# Autodesk Inventor assembly: Cartesian2_YAssembly
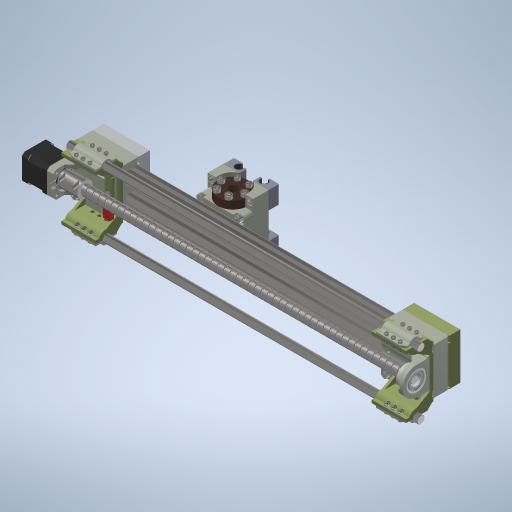
[picture p0: Inventor's stored thumbnail of the model, 512x512]
Saved by Autodesk Inventor 2024 (Build 280153000, 153)
## iProperties
Created: 2020-08-17
Part Number: Cartesian2_YAssembly
Material: Ogólny
Document SubType Name: Assembly
Designer: invin
Mass: 4227.11 g
Surface Area: 5602.37 cm^2
Volume: 1262.4 cm^3
Density: 3.34848 g/cm^3
Author: invin
## Documents named in this file (27)
- D:\@home\mikoma\Dokumenty\DR\CartesianRobotsDigitalTwin\model\Workspaces\Obszar roboczy\assembly_v3\Y\Y.iam
- D:\@home\mikoma\Dokumenty\DR\CartesianRobotsDigitalTwin\model\Workspaces\Obszar roboczy\content\item\item_0037003_Profile_5_20x20_L=564_1.ipt
- D:\@home\mikoma\Dokumenty\DR\CartesianRobotsDigitalTwin\model\Workspaces\Obszar roboczy\content\manipulatorSharedParts\Cartesian1_12mm_Rod.ipt
- D:\@home\mikoma\Dokumenty\DR\CartesianRobotsDigitalTwin\model\Workspaces\Obszar roboczy\content\manipulatorSharedParts\Cartesian2_BallBearing_25x37x7.ipt
- D:\@home\mikoma\Dokumenty\DR\CartesianRobotsDigitalTwin\model\Workspaces\Obszar roboczy\assembly_v3\Y\Cartesian1_X_RodCover.ipt
- D:\@home\mikoma\Dokumenty\DR\CartesianRobotsDigitalTwin\model\Workspaces\Obszar roboczy\content\nema17\Nema17 Stepper Motor.ipt
- D:\@home\mikoma\Dokumenty\DR\CartesianRobotsDigitalTwin\model\Workspaces\Obszar roboczy\content\manipulatorSharedParts\Cartesian1_12_12_Clutch.ipt
- D:\@home\mikoma\Dokumenty\DR\CartesianRobotsDigitalTwin\model\Workspaces\Obszar roboczy\content\manipulatorSharedParts\Cartesian1_BallScrew.ipt
- D:\@home\mikoma\Dokumenty\DR\CartesianRobotsDigitalTwin\model\Workspaces\Obszar roboczy\content\igus\WJ200UM_01_10_1.ipt
- D:\@home\mikoma\Dokumenty\DR\CartesianRobotsDigitalTwin\model\Workspaces\Obszar roboczy\assembly_v3\Y\YSub1.iam
- D:\@home\mikoma\Dokumenty\DR\CartesianRobotsDigitalTwin\model\Workspaces\Obszar roboczy\assembly_v3\Y\YSub2.iam
- D:\@home\mikoma\Dokumenty\DR\CartesianRobotsDigitalTwin\model\Workspaces\Obszar roboczy\assembly_v3\Y\YItemEndCover.ipt
- D:\@home\mikoma\Dokumenty\DR\CartesianRobotsDigitalTwin\model\Workspaces\Obszar roboczy\assembly_v3\Y\YCarriage.ipt
- D:\@home\mikoma\Dokumenty\DR\CartesianRobotsDigitalTwin\model\Workspaces\Obszar roboczy\assembly_v3\Y\YCarriageNut.ipt
- D:\@home\mikoma\Dokumenty\DR\CartesianRobotsDigitalTwin\model\Workspaces\Obszar roboczy\assembly_v3\Y\YItemEnd.ipt
- D:\@home\mikoma\Dokumenty\DR\CartesianRobotsDigitalTwin\model\Workspaces\Obszar roboczy\assembly_v3\Y\YItemEndCoverConnector.ipt
- D:\@home\mikoma\Dokumenty\DR\CartesianRobotsDigitalTwin\model\Workspaces\Obszar roboczy\content\manipulatorSharedParts\endCup.ipt
- D:\@home\mikoma\Dokumenty\DR\CartesianRobotsDigitalTwin\model\Workspaces\Obszar roboczy\CC\pl-PL\ISO 4762(1)\DIN EN ISO 4762 - M5 x 50.ipt
- D:\@home\mikoma\Dokumenty\DR\CartesianRobotsDigitalTwin\model\Workspaces\Obszar roboczy\CC\pl-PL\ISO 4762(1)\DIN EN ISO 4762 - M6 x 55.ipt
- D:\@home\mikoma\Dokumenty\DR\CartesianRobotsDigitalTwin\model\Workspaces\Obszar roboczy\CC\pl-PL\ISO 4032(2)\ISO 4032 - M6 - ISO.ipt
- D:\@home\mikoma\Dokumenty\DR\CartesianRobotsDigitalTwin\model\Workspaces\Obszar roboczy\CC\pl-PL\ISO 4762(1)\DIN EN ISO 4762 - M6 x 30.ipt
- D:\@home\mikoma\Dokumenty\DR\CartesianRobotsDigitalTwin\model\Workspaces\Obszar roboczy\content\item\item_0037006_Wpust_przesuwny_5_St_M4_1.ipt
- D:\@home\mikoma\Dokumenty\DR\CartesianRobotsDigitalTwin\model\Workspaces\Obszar roboczy\CC\pl-PL\DIN 7984\DIN 7984 - M4 x 14.ipt
- D:\@home\mikoma\Dokumenty\DR\CartesianRobotsDigitalTwin\model\Workspaces\Obszar roboczy\CC\pl-PL\ISO 4032(2)\ISO 4032 - M5 - ISO.ipt
- D:\@home\mikoma\Dokumenty\DR\CartesianRobotsDigitalTwin\model\Workspaces\Obszar roboczy\content\manipulatorSharedParts\Connector_female.ipt
- D:\@home\mikoma\Dokumenty\DR\CartesianRobotsDigitalTwin\model\Workspaces\Obszar roboczy\CC\pl-PL\ISO 4032(2)\ISO 4032 - M3 - ISO.ipt
- D:\@home\mikoma\Dokumenty\DR\CartesianRobotsDigitalTwin\model\Workspaces\Obszar roboczy\CC\pl-PL\ISO 4762(1)\DIN EN ISO 4762 - M3 x 12.ipt
## Components (115 placed, 26 different names)
1. YSub1:1 [sub-assembly] — Zestawiający:1, Kąt:1, Zestawiający:6, Zestawiający:7, Zestawiający:9, Zestawiający:10, Zestawiający:13, Zestawiający:32, Zestawiający:33, Zestawiający:34, Zestawiający:35, Zestawiający:36, Zestawiający:37, Zestawiający:44, Kąt:3, Zestawiający:45, Zestawiające:57, Zestawiające:75, Równoległe:14, Równoległe:15, Zestawiające:82, Zestawiające:83, Zestawiające:84, Zestawiające:85, Zestawiające:86, Zestawiające:87, Zestawiające:88, Zestawiające:89, Zestawiające:90, Równoległe:20, Równoległe:21, Zestawiające:174, Zestawiające:179, Kątowe:21, Kątowe:24
2. YSub2:1 [sub-assembly] — Zestawiający:1, Kąt:1, Zestawiający:12, Zestawiający:24, Zestawiający:25, Zestawiający:26, Zestawiający:27, Zestawiający:28, Zestawiający:29, Zestawiający:30, Zestawiający:31, Zestawiające:50, Równoległe:3, Zestawiające:91, Zestawiające:92, Zestawiające:93, Zestawiające:94, Zestawiające:95, Zestawiające:96, Zestawiające:97, Zestawiające:98, Zestawiające:184, Kątowe:22, Zestawiające:188, Kątowe:23
3. YItemEnd:1 — Zestawiające:50, Zestawiające:52, Równoległe:3, Zestawiające:53, Równoległe:4, Równoległe:5, Zestawiające:55, Zestawiające:56
4. item_0037003_Profile_5_20x20_L=564_1:1 — Zestawiający:9, Zestawiający:10, Zestawiające:56, Kątowe:10, Zestawiające:145, Kątowe:11, Zestawiające:149
5. item_0037003_Profile_5_20x20_L=564_1:2 — Zestawiający:6, Zestawiający:7, Zestawiające:52, Zestawiające:55, Zestawiające:57, Zestawiające:58, Zestawiające:138, Kątowe:8, Kątowe:9, Zestawiające:141
6. Cartesian1_12mm_Rod:1 — Zestawiający:13, Równoległe:21
7. Cartesian1_12mm_Rod:2 — Zestawiający:12, Równoległe:20
8. Cartesian2_BallBearing_25x37x7:1 — Zestawiający:24, Zestawiający:25, Zestawiające:78, Zestawiające:80, Zestawiające:81
9. Cartesian1_X_RodCover:1 — Zestawiający:26, Zestawiający:27, Zestawiający:28, Zestawiające:181, Zestawiające:182
10. Cartesian1_X_RodCover:2 — Zestawiający:29, Zestawiający:30, Zestawiający:31, Zestawiające:186, Zestawiające:187
11. Cartesian1_X_RodCover:3 — Zestawiający:32, Zestawiający:33, Zestawiający:34
12. Cartesian1_X_RodCover:4 — Zestawiający:35, Zestawiający:36, Zestawiający:37, Zestawiające:176, Zestawiające:177
13. Nema17 Stepper Motor:2 — Zestawiający:44, Kąt:3, Zestawiający:45, Zestawiający:46, Zestawiający:47
14. Cartesian1_12_12_Clutch:1 — Zestawiający:46, Zestawiający:47, Zestawiający:48, Zestawiający:49
15. Cartesian1_BallScrew:1 — Zestawiający:48, Zestawiający:49
16. YItemEndCover:1 — Zestawiające:53, Równoległe:4, Równoległe:5, Kątowe:12, Zestawiające:153, Kątowe:13, Zestawiające:155, Kątowe:14, Zestawiające:157, Kątowe:15, Zestawiające:159
17. YCarriage:1 — Zestawiające:58, Zestawiające:59, Zestawiające:61, Zestawiające:62, Zestawiające:63, Zestawiające:64, Zestawiające:65, Zestawiające:66, Zestawiające:67, Zestawiające:68, Zestawiające:69, Zestawiające:70, Zestawiające:71, Zestawiające:72, Zestawiające:73, Równoległe:13, Zestawiające:99, Zestawiające:111, Zestawiające:112, Zestawiające:113, Zestawiające:114, Zestawiające:115, Zestawiające:116, Zestawiające:117, Zestawiające:118, Zestawiające:119, Zestawiające:120, Zestawiające:121, Zestawiające:122, Zestawiające:123, Kątowe:4, Zestawiające:125, Zestawiające:127, Kątowe:5, Kątowe:6, Zestawiające:128, Kątowe:7, Zestawiające:130, Zestawiające:132, Zestawiające:133, Zestawiające:134, Zestawiające:135, Zestawiające:136, Zestawiające:137, Zestawiające:139, Zestawiające:140, Zestawiające:142, Zestawiające:143, Zestawiające:144, Zestawiające:146, Zestawiające:147, Zestawiające:148, Zestawiające:150, Zestawiające:151
18. YCarriageNut:1 — Zestawiające:59, Zestawiające:61, Zestawiające:82, Zestawiające:100, Zestawiające:101, Zestawiające:102, Zestawiające:103, Zestawiające:104, Zestawiające:105, Zestawiające:106, Zestawiające:107, Zestawiające:108, Zestawiające:109, Zestawiające:110
19. WJ200UM_01_10_1:1 — Zestawiające:62, Zestawiające:63, Zestawiające:64
20. WJ200UM_01_10_1:2 — Zestawiające:65, Zestawiające:66, Zestawiające:67
21. WJ200UM_01_10_1:3 — Zestawiające:68, Zestawiające:69, Zestawiające:70
22. WJ200UM_01_10_1:4 — Zestawiające:71, Zestawiające:72, Zestawiające:73
23. YItemEndCoverConnector:1 — Zestawiające:75, Równoległe:14, Równoległe:15, Zestawiające:79, Kątowe:16, Zestawiające:161, Kątowe:17, Zestawiające:163, Kątowe:18, Zestawiające:165, Kątowe:19, Zestawiające:167, Zestawiające:168, Zestawiające:169, Zestawiające:170
24. endCup:1 — Zestawiające:80, Zestawiające:81
25. DIN EN ISO 4762 M5 x 50:1 — Zestawiające:83, Zestawiające:84, Zestawiające:160
26. DIN EN ISO 4762 M5 x 50:2 — Zestawiające:85, Zestawiające:86, Zestawiające:166
27. DIN EN ISO 4762 M5 x 50:3 — Zestawiające:87, Zestawiające:88, Zestawiające:162
28. DIN EN ISO 4762 M5 x 50:4 — Zestawiające:89, Zestawiające:90, Zestawiające:164
29. DIN EN ISO 4762 M5 x 50:5 — Zestawiające:91, Zestawiające:95, Zestawiające:152
30. DIN EN ISO 4762 M5 x 50:6 — Zestawiające:92, Zestawiające:98, Zestawiające:158
31. DIN EN ISO 4762 M5 x 50:7 — Zestawiające:93, Zestawiające:96, Zestawiające:154
32. DIN EN ISO 4762 M5 x 50:8 — Zestawiające:94, Zestawiające:97, Zestawiające:156
33. DIN EN ISO 4762 M5 x 50:9 — Zestawiające:99, Zestawiające:100
34. DIN EN ISO 4762 M5 x 50:10 — Zestawiające:101, Zestawiające:102
35. DIN EN ISO 4762 M6 x 55:1 — Zestawiające:103, Zestawiające:107, Zestawiające:131
36. DIN EN ISO 4762 M6 x 55:2 — Zestawiające:111, Zestawiające:112
37. DIN EN ISO 4762 M6 x 55:3 — Zestawiające:104, Zestawiające:108, Zestawiające:129
38. DIN EN ISO 4762 M6 x 55:4 — Zestawiające:105, Zestawiające:110, Zestawiające:124
39. DIN EN ISO 4762 M6 x 55:5 — Zestawiające:106, Zestawiające:109, Zestawiające:123, Zestawiające:126
40. DIN EN ISO 4762 M6 x 55:6 — Zestawiające:113, Zestawiające:114
41. DIN EN ISO 4762 M6 x 55:7 — Zestawiające:115, Zestawiające:116
42. DIN EN ISO 4762 M6 x 55:8 — Zestawiające:117, Zestawiające:118
43. DIN EN ISO 4762 M6 x 55:9 — Zestawiające:119, Zestawiające:120
44. DIN EN ISO 4762 M6 x 55:10 — Zestawiające:121, Zestawiające:122
45. ISO 4032 M6:1 — Zestawiające:124, Kątowe:4, Zestawiające:125
46. ISO 4032 M6:2 — Zestawiające:126, Zestawiające:127, Kątowe:5
47. ISO 4032 M6:3 — Kątowe:6, Zestawiające:128, Zestawiające:129
48. ISO 4032 M6:4 — Kątowe:7, Zestawiające:130, Zestawiające:131
49. DIN EN ISO 4762 M6 x 30:1 — Zestawiające:132, Zestawiające:133
50. DIN EN ISO 4762 M6 x 30:2 — Zestawiające:134, Zestawiające:135
51. item_0037006_Wpust_przesuwny_5_St_M4_1:1 — Zestawiające:137, Zestawiające:138, Kątowe:8
52. DIN 7984 M4 x 14:1 — Zestawiające:136, Zestawiające:139
53. DIN 7984 M4 x 14:2 — Zestawiające:142, Zestawiające:143
54. item_0037006_Wpust_przesuwny_5_St_M4_1:2 — Zestawiające:140, Kątowe:9, Zestawiające:141
55. item_0037006_Wpust_przesuwny_5_St_M4_1:3 — Zestawiające:144, Kątowe:10, Zestawiające:145
56. DIN 7984 M4 x 14:3 — Zestawiające:146, Zestawiające:147
57. item_0037006_Wpust_przesuwny_5_St_M4_1:4 — Zestawiające:148, Kątowe:11, Zestawiające:149
58. DIN 7984 M4 x 14:4 — Zestawiające:150, Zestawiające:151
59. ISO 4032 M5:1 — Zestawiające:152, Kątowe:12, Zestawiające:153
60. ISO 4032 M5:2 — Zestawiające:154, Kątowe:13, Zestawiające:155
61. ISO 4032 M5:3 — Zestawiające:156, Kątowe:14, Zestawiające:157
62. ISO 4032 M5:4 — Zestawiające:158, Kątowe:15, Zestawiające:159
63. ISO 4032 M5:5 — Zestawiające:160, Kątowe:16, Zestawiające:161
64. ISO 4032 M5:6 — Zestawiające:162, Kątowe:17, Zestawiające:163
65. ISO 4032 M5:7 — Zestawiające:164, Kątowe:18, Zestawiające:165
66. ISO 4032 M5:8 — Zestawiające:166, Kątowe:19, Zestawiające:167
67. Connector_female:1 — Zestawiające:168, Zestawiające:169, Zestawiające:170
68. DIN EN ISO 4762 M3 x 12:1
69. ISO 4032 M3:1 — Zestawiające:174, Kątowe:24
70. DIN EN ISO 4762 M3 x 12:2
71. ISO 4032 M3:2
72. DIN EN ISO 4762 M3 x 12:3
73. ISO 4032 M3:3
74. DIN EN ISO 4762 M3 x 12:4
75. ISO 4032 M3:4
76. DIN EN ISO 4762 M3 x 12:5
77. ISO 4032 M3:5
78. DIN EN ISO 4762 M3 x 12:6
79. ISO 4032 M3:6
80. DIN EN ISO 4762 M3 x 12:7 — Zestawiające:176, Zestawiające:177, Zestawiające:178
81. ISO 4032 M3:7 — Zestawiające:178, Zestawiające:179, Kątowe:21
82. DIN EN ISO 4762 M3 x 12:8
83. ISO 4032 M3:8
84. DIN EN ISO 4762 M3 x 12:9
85. ISO 4032 M3:9
86. DIN EN ISO 4762 M3 x 12:10
87. ISO 4032 M3:10
88. DIN EN ISO 4762 M3 x 12:11
89. ISO 4032 M3:11
90. DIN EN ISO 4762 M3 x 12:12
91. ISO 4032 M3:12
92. ISO 4032 M3:13 — Zestawiające:183, Zestawiające:184, Kątowe:22
93. DIN EN ISO 4762 M3 x 12:13 — Zestawiające:181, Zestawiające:182, Zestawiające:183
94. ISO 4032 M3:14
95. DIN EN ISO 4762 M3 x 12:14
96. ISO 4032 M3:15
97. DIN EN ISO 4762 M3 x 12:15
98. ISO 4032 M3:16
99. DIN EN ISO 4762 M3 x 12:16
100. ISO 4032 M3:17
101. DIN EN ISO 4762 M3 x 12:17
102. ISO 4032 M3:18
103. DIN EN ISO 4762 M3 x 12:18
104. DIN EN ISO 4762 M3 x 12:19 — Zestawiające:186, Zestawiające:187
105. ISO 4032 M3:19 — Zestawiające:188, Kątowe:23
106. DIN EN ISO 4762 M3 x 12:20
107. ISO 4032 M3:20
108. DIN EN ISO 4762 M3 x 12:21
109. ISO 4032 M3:21
110. DIN EN ISO 4762 M3 x 12:22
111. ISO 4032 M3:22
112. DIN EN ISO 4762 M3 x 12:23
113. ISO 4032 M3:23
114. DIN EN ISO 4762 M3 x 12:24
115. ISO 4032 M3:24
## Component patterns: (6 elements, first: DIN EN ISO 4762 M3 x 12:1 + ISO 4032 M3:1), (6 elements, first: DIN EN ISO 4762 M3 x 12:7 + ISO 4032 M3:7), (6 elements, first: ISO 4032 M3:13 + DIN EN ISO 4762 M3 x 12:13), (6 elements, first: DIN EN ISO 4762 M3 x 12:19 + ISO 4032 M3:19)
## Relationships (190: Mate 160, Angle 22, Flush 8)
- Zestawiający:1 [Mate]: YSub1:1 ↔ YSub2:1
- Kąt:1 [Angle] (0 deg): YSub1:1 ↔ YSub2:1
- Zestawiający:6 [Mate]: YSub1:1 ↔ item_0037003_Profile_5_20x20_L=564_1:2
- Zestawiający:7 [Mate]: YSub1:1 ↔ item_0037003_Profile_5_20x20_L=564_1:2
- Zestawiający:9 [Mate]: YSub1:1 ↔ item_0037003_Profile_5_20x20_L=564_1:1
- Zestawiający:10 [Mate]: YSub1:1 ↔ item_0037003_Profile_5_20x20_L=564_1:1
- Zestawiający:12 [Mate]: YSub2:1 ↔ Cartesian1_12mm_Rod:2
- Zestawiający:13 [Mate]: YSub1:1 ↔ Cartesian1_12mm_Rod:1
- Zestawiający:24 [Mate]: YSub2:1 ↔ Cartesian2_BallBearing_25x37x7:1
- Zestawiający:25 [Mate]: YSub2:1 ↔ Cartesian2_BallBearing_25x37x7:1
- Zestawiający:26 [Mate]: YSub2:1 ↔ Cartesian1_X_RodCover:1
- Zestawiający:27 [Mate]: YSub2:1 ↔ Cartesian1_X_RodCover:1
- Zestawiający:28 [Mate]: YSub2:1 ↔ Cartesian1_X_RodCover:1
- Zestawiający:29 [Mate]: YSub2:1 ↔ Cartesian1_X_RodCover:2
- Zestawiający:30 [Mate]: YSub2:1 ↔ Cartesian1_X_RodCover:2
- Zestawiający:31 [Mate]: YSub2:1 ↔ Cartesian1_X_RodCover:2
- Zestawiający:32 [Mate]: YSub1:1 ↔ Cartesian1_X_RodCover:3
- Zestawiający:33 [Mate]: YSub1:1 ↔ Cartesian1_X_RodCover:3
- Zestawiający:34 [Mate]: YSub1:1 ↔ Cartesian1_X_RodCover:3
- Zestawiający:35 [Mate]: YSub1:1 ↔ Cartesian1_X_RodCover:4
- Zestawiający:36 [Mate]: YSub1:1 ↔ Cartesian1_X_RodCover:4
- Zestawiający:37 [Mate]: YSub1:1 ↔ Cartesian1_X_RodCover:4
- Zestawiający:44 [Mate]: YSub1:1 ↔ Nema17 Stepper Motor:2
- Kąt:3 [Angle] (0 deg): YSub1:1 ↔ Nema17 Stepper Motor:2
- Zestawiający:45 [Mate]: YSub1:1 ↔ Nema17 Stepper Motor:2
- Zestawiający:46 [Mate]: Nema17 Stepper Motor:2 ↔ Cartesian1_12_12_Clutch:1
- Zestawiający:47 [Mate] (6 mm): Nema17 Stepper Motor:2 ↔ Cartesian1_12_12_Clutch:1
- Zestawiający:48 [Mate]: Cartesian1_12_12_Clutch:1 ↔ Cartesian1_BallScrew:1
- Zestawiający:49 [Mate]: Cartesian1_12_12_Clutch:1 ↔ Cartesian1_BallScrew:1
- Zestawiające:50 [Mate]: YSub2:1 ↔ YItemEnd:1
- Zestawiające:52 [Mate]: YItemEnd:1 ↔ item_0037003_Profile_5_20x20_L=564_1:2
- Równoległe:3 [Flush]: YSub2:1 ↔ YItemEnd:1
- Zestawiające:53 [Mate]: YItemEnd:1 ↔ YItemEndCover:1
- Równoległe:4 [Flush]: YItemEnd:1 ↔ YItemEndCover:1
- Równoległe:5 [Flush]: YItemEnd:1 ↔ YItemEndCover:1
- Zestawiające:55 [Mate]: YItemEnd:1 ↔ item_0037003_Profile_5_20x20_L=564_1:2
- Zestawiające:56 [Mate]: YItemEnd:1 ↔ item_0037003_Profile_5_20x20_L=564_1:1
- Zestawiające:57 [Mate]: YSub1:1 ↔ item_0037003_Profile_5_20x20_L=564_1:2
- Zestawiające:58 [Mate]: item_0037003_Profile_5_20x20_L=564_1:2 ↔ YCarriage:1
- Zestawiające:59 [Mate]: YCarriage:1 ↔ YCarriageNut:1
- Zestawiające:61 [Mate]: YCarriage:1 ↔ YCarriageNut:1
- Zestawiające:62 [Mate]: YCarriage:1 ↔ WJ200UM_01_10_1:1
- Zestawiające:63 [Mate]: YCarriage:1 ↔ WJ200UM_01_10_1:1
- Zestawiające:64 [Mate]: YCarriage:1 ↔ WJ200UM_01_10_1:1
- Zestawiające:65 [Mate]: YCarriage:1 ↔ WJ200UM_01_10_1:2
- Zestawiające:66 [Mate]: YCarriage:1 ↔ WJ200UM_01_10_1:2
- Zestawiające:67 [Mate]: YCarriage:1 ↔ WJ200UM_01_10_1:2
- Zestawiające:68 [Mate]: YCarriage:1 ↔ WJ200UM_01_10_1:3
- Zestawiające:69 [Mate]: YCarriage:1 ↔ WJ200UM_01_10_1:3
- Zestawiające:70 [Mate]: YCarriage:1 ↔ WJ200UM_01_10_1:3
- Zestawiające:71 [Mate]: YCarriage:1 ↔ WJ200UM_01_10_1:4
- Zestawiające:72 [Mate]: YCarriage:1 ↔ WJ200UM_01_10_1:4
- Zestawiające:73 [Mate]: YCarriage:1 ↔ WJ200UM_01_10_1:4
- Równoległe:13 [Flush]: YCarriage:1
- Zestawiające:75 [Mate]: YSub1:1 ↔ YItemEndCoverConnector:1
- Równoległe:14 [Flush]: YSub1:1 ↔ YItemEndCoverConnector:1
- Równoległe:15 [Flush]: YSub1:1 ↔ YItemEndCoverConnector:1
- Zestawiające:78 [Mate]: Cartesian2_BallBearing_25x37x7:1
- Zestawiające:79 [Mate]: YItemEndCoverConnector:1
- Zestawiające:80 [Mate]: Cartesian2_BallBearing_25x37x7:1 ↔ endCup:1
- Zestawiające:81 [Mate]: Cartesian2_BallBearing_25x37x7:1 ↔ endCup:1
- Zestawiające:82 [Mate] (-201 mm): YSub1:1 ↔ YCarriageNut:1
- Zestawiające:83 [Mate]: YSub1:1 ↔ DIN EN ISO 4762 M5 x 50:1
- Zestawiające:84 [Mate]: YSub1:1 ↔ DIN EN ISO 4762 M5 x 50:1
- Zestawiające:85 [Mate]: YSub1:1 ↔ DIN EN ISO 4762 M5 x 50:2
- Zestawiające:86 [Mate]: YSub1:1 ↔ DIN EN ISO 4762 M5 x 50:2
- Zestawiające:87 [Mate]: YSub1:1 ↔ DIN EN ISO 4762 M5 x 50:3
- Zestawiające:88 [Mate] (-4 mm): YSub1:1 ↔ DIN EN ISO 4762 M5 x 50:3
- Zestawiające:89 [Mate]: YSub1:1 ↔ DIN EN ISO 4762 M5 x 50:4
- Zestawiające:90 [Mate] (-4 mm): YSub1:1 ↔ DIN EN ISO 4762 M5 x 50:4
- Zestawiające:91 [Mate]: YSub2:1 ↔ DIN EN ISO 4762 M5 x 50:5
- Zestawiające:92 [Mate]: YSub2:1 ↔ DIN EN ISO 4762 M5 x 50:6
- Zestawiające:93 [Mate]: YSub2:1 ↔ DIN EN ISO 4762 M5 x 50:7
- Zestawiające:94 [Mate]: YSub2:1 ↔ DIN EN ISO 4762 M5 x 50:8
- Zestawiające:95 [Mate]: YSub2:1 ↔ DIN EN ISO 4762 M5 x 50:5
- Zestawiające:96 [Mate]: YSub2:1 ↔ DIN EN ISO 4762 M5 x 50:7
- Zestawiające:97 [Mate]: YSub2:1 ↔ DIN EN ISO 4762 M5 x 50:8
- Zestawiające:98 [Mate]: YSub2:1 ↔ DIN EN ISO 4762 M5 x 50:6
- Równoległe:20 [Flush] (-4 mm): YSub1:1 ↔ Cartesian1_12mm_Rod:2
- Równoległe:21 [Flush] (-4 mm): YSub1:1 ↔ Cartesian1_12mm_Rod:1
- Zestawiające:99 [Mate]: YCarriage:1 ↔ DIN EN ISO 4762 M5 x 50:9
- Zestawiające:100 [Mate]: YCarriageNut:1 ↔ DIN EN ISO 4762 M5 x 50:9
- Zestawiające:101 [Mate]: YCarriageNut:1 ↔ DIN EN ISO 4762 M5 x 50:10
- Zestawiające:102 [Mate]: YCarriageNut:1 ↔ DIN EN ISO 4762 M5 x 50:10
- Zestawiające:103 [Mate]: YCarriageNut:1 ↔ DIN EN ISO 4762 M6 x 55:1
- Zestawiające:104 [Mate]: YCarriageNut:1 ↔ DIN EN ISO 4762 M6 x 55:3
- Zestawiające:105 [Mate]: YCarriageNut:1 ↔ DIN EN ISO 4762 M6 x 55:4
- Zestawiające:106 [Mate]: YCarriageNut:1 ↔ DIN EN ISO 4762 M6 x 55:5
- Zestawiające:107 [Mate]: YCarriageNut:1 ↔ DIN EN ISO 4762 M6 x 55:1
- Zestawiające:108 [Mate]: YCarriageNut:1 ↔ DIN EN ISO 4762 M6 x 55:3
- Zestawiające:109 [Mate]: YCarriageNut:1 ↔ DIN EN ISO 4762 M6 x 55:5
- Zestawiające:110 [Mate]: YCarriageNut:1 ↔ DIN EN ISO 4762 M6 x 55:4
- Zestawiające:111 [Mate]: YCarriage:1 ↔ DIN EN ISO 4762 M6 x 55:2
- Zestawiające:112 [Mate]: YCarriage:1 ↔ DIN EN ISO 4762 M6 x 55:2
- Zestawiające:113 [Mate]: YCarriage:1 ↔ DIN EN ISO 4762 M6 x 55:6
- Zestawiające:114 [Mate]: YCarriage:1 ↔ DIN EN ISO 4762 M6 x 55:6
- Zestawiające:115 [Mate]: YCarriage:1 ↔ DIN EN ISO 4762 M6 x 55:7
- Zestawiające:116 [Mate]: YCarriage:1 ↔ DIN EN ISO 4762 M6 x 55:7
- Zestawiające:117 [Mate]: YCarriage:1 ↔ DIN EN ISO 4762 M6 x 55:8
- Zestawiające:118 [Mate]: YCarriage:1 ↔ DIN EN ISO 4762 M6 x 55:8
- Zestawiające:119 [Mate]: YCarriage:1 ↔ DIN EN ISO 4762 M6 x 55:9
- Zestawiające:120 [Mate]: YCarriage:1 ↔ DIN EN ISO 4762 M6 x 55:9
- Zestawiające:121 [Mate]: YCarriage:1 ↔ DIN EN ISO 4762 M6 x 55:10
- Zestawiające:122 [Mate]: YCarriage:1 ↔ DIN EN ISO 4762 M6 x 55:10
- Zestawiające:123 [Mate]: YCarriage:1 ↔ DIN EN ISO 4762 M6 x 55:5
- Zestawiające:124 [Mate]: DIN EN ISO 4762 M6 x 55:4 ↔ ISO 4032 M6:1
- Kątowe:4 [Angle] (0 deg): YCarriage:1 ↔ ISO 4032 M6:1
- Zestawiające:125 [Mate]: YCarriage:1 ↔ ISO 4032 M6:1
- Zestawiające:126 [Mate]: DIN EN ISO 4762 M6 x 55:5 ↔ ISO 4032 M6:2
- Zestawiające:127 [Mate]: YCarriage:1 ↔ ISO 4032 M6:2
- Kątowe:5 [Angle] (0 deg): YCarriage:1 ↔ ISO 4032 M6:2
- Kątowe:6 [Angle] (0 deg): YCarriage:1 ↔ ISO 4032 M6:3
- Zestawiające:128 [Mate]: YCarriage:1 ↔ ISO 4032 M6:3
- Zestawiające:129 [Mate]: DIN EN ISO 4762 M6 x 55:3 ↔ ISO 4032 M6:3
- Kątowe:7 [Angle] (0 deg): YCarriage:1 ↔ ISO 4032 M6:4
- Zestawiające:130 [Mate]: YCarriage:1 ↔ ISO 4032 M6:4
- Zestawiające:131 [Mate]: DIN EN ISO 4762 M6 x 55:1 ↔ ISO 4032 M6:4
- Zestawiające:132 [Mate]: YCarriage:1 ↔ DIN EN ISO 4762 M6 x 30:1
- Zestawiające:133 [Mate]: YCarriage:1 ↔ DIN EN ISO 4762 M6 x 30:1
- Zestawiające:134 [Mate]: YCarriage:1 ↔ DIN EN ISO 4762 M6 x 30:2
- Zestawiające:135 [Mate]: YCarriage:1 ↔ DIN EN ISO 4762 M6 x 30:2
- Zestawiające:136 [Mate]: YCarriage:1 ↔ DIN 7984 M4 x 14:1
- Zestawiające:137 [Mate]: YCarriage:1 ↔ item_0037006_Wpust_przesuwny_5_St_M4_1:1
- Zestawiające:138 [Mate]: item_0037003_Profile_5_20x20_L=564_1:2 ↔ item_0037006_Wpust_przesuwny_5_St_M4_1:1
- Kątowe:8 [Angle] (0 deg): item_0037003_Profile_5_20x20_L=564_1:2 ↔ item_0037006_Wpust_przesuwny_5_St_M4_1:1
- Zestawiające:139 [Mate]: YCarriage:1 ↔ DIN 7984 M4 x 14:1
- Zestawiające:140 [Mate]: YCarriage:1 ↔ item_0037006_Wpust_przesuwny_5_St_M4_1:2
- Kątowe:9 [Angle] (180 deg): item_0037003_Profile_5_20x20_L=564_1:2 ↔ item_0037006_Wpust_przesuwny_5_St_M4_1:2
- Zestawiające:141 [Mate]: item_0037003_Profile_5_20x20_L=564_1:2 ↔ item_0037006_Wpust_przesuwny_5_St_M4_1:2
- Zestawiające:142 [Mate]: YCarriage:1 ↔ DIN 7984 M4 x 14:2
- Zestawiające:143 [Mate]: YCarriage:1 ↔ DIN 7984 M4 x 14:2
- Zestawiające:144 [Mate]: YCarriage:1 ↔ item_0037006_Wpust_przesuwny_5_St_M4_1:3
- Kątowe:10 [Angle] (0 deg): item_0037003_Profile_5_20x20_L=564_1:1 ↔ item_0037006_Wpust_przesuwny_5_St_M4_1:3
- Zestawiające:145 [Mate]: item_0037003_Profile_5_20x20_L=564_1:1 ↔ item_0037006_Wpust_przesuwny_5_St_M4_1:3
- Zestawiające:146 [Mate]: YCarriage:1 ↔ DIN 7984 M4 x 14:3
- Zestawiające:147 [Mate]: YCarriage:1 ↔ DIN 7984 M4 x 14:3
- Zestawiające:148 [Mate]: YCarriage:1 ↔ item_0037006_Wpust_przesuwny_5_St_M4_1:4
- Kątowe:11 [Angle] (180 deg): item_0037003_Profile_5_20x20_L=564_1:1 ↔ item_0037006_Wpust_przesuwny_5_St_M4_1:4
- Zestawiające:149 [Mate]: item_0037003_Profile_5_20x20_L=564_1:1 ↔ item_0037006_Wpust_przesuwny_5_St_M4_1:4
- Zestawiające:150 [Mate]: YCarriage:1 ↔ DIN 7984 M4 x 14:4
- Zestawiające:151 [Mate]: YCarriage:1 ↔ DIN 7984 M4 x 14:4
- Zestawiające:152 [Mate]: DIN EN ISO 4762 M5 x 50:5 ↔ ISO 4032 M5:1
- Kątowe:12 [Angle] (0 deg): YItemEndCover:1 ↔ ISO 4032 M5:1
- Zestawiające:153 [Mate]: YItemEndCover:1 ↔ ISO 4032 M5:1
- Zestawiające:154 [Mate]: DIN EN ISO 4762 M5 x 50:7 ↔ ISO 4032 M5:2
- Kątowe:13 [Angle] (0 deg): YItemEndCover:1 ↔ ISO 4032 M5:2
- Zestawiające:155 [Mate]: YItemEndCover:1 ↔ ISO 4032 M5:2
- Zestawiające:156 [Mate]: DIN EN ISO 4762 M5 x 50:8 ↔ ISO 4032 M5:3
- Kątowe:14 [Angle] (0 deg): YItemEndCover:1 ↔ ISO 4032 M5:3
- Zestawiające:157 [Mate]: YItemEndCover:1 ↔ ISO 4032 M5:3
- Zestawiające:158 [Mate]: DIN EN ISO 4762 M5 x 50:6 ↔ ISO 4032 M5:4
- Kątowe:15 [Angle] (0 deg): YItemEndCover:1 ↔ ISO 4032 M5:4
- Zestawiające:159 [Mate]: YItemEndCover:1 ↔ ISO 4032 M5:4
- Zestawiające:160 [Mate]: DIN EN ISO 4762 M5 x 50:1 ↔ ISO 4032 M5:5
- Kątowe:16 [Angle] (0 deg): YItemEndCoverConnector:1 ↔ ISO 4032 M5:5
- Zestawiające:161 [Mate]: YItemEndCoverConnector:1 ↔ ISO 4032 M5:5
- Zestawiające:162 [Mate]: DIN EN ISO 4762 M5 x 50:3 ↔ ISO 4032 M5:6
- Kątowe:17 [Angle] (0 deg): YItemEndCoverConnector:1 ↔ ISO 4032 M5:6
- Zestawiające:163 [Mate]: YItemEndCoverConnector:1 ↔ ISO 4032 M5:6
- Zestawiające:164 [Mate]: DIN EN ISO 4762 M5 x 50:4 ↔ ISO 4032 M5:7
- Kątowe:18 [Angle] (0 deg): YItemEndCoverConnector:1 ↔ ISO 4032 M5:7
- Zestawiające:165 [Mate]: YItemEndCoverConnector:1 ↔ ISO 4032 M5:7
- Zestawiające:166 [Mate]: DIN EN ISO 4762 M5 x 50:2 ↔ ISO 4032 M5:8
- Kątowe:19 [Angle] (0 deg): YItemEndCoverConnector:1 ↔ ISO 4032 M5:8
- Zestawiające:167 [Mate]: YItemEndCoverConnector:1 ↔ ISO 4032 M5:8
- Zestawiające:168 [Mate]: YItemEndCoverConnector:1 ↔ Connector_female:1
- Zestawiające:169 [Mate]: YItemEndCoverConnector:1 ↔ Connector_female:1
- Zestawiające:170 [Mate]: YItemEndCoverConnector:1 ↔ Connector_female:1
- [Mate]: Cartesian1_X_RodCover:3 ↔ DIN EN ISO 4762 M3 x 12:1
- [Mate]: Cartesian1_X_RodCover:3 ↔ DIN EN ISO 4762 M3 x 12:1
- [Mate]: DIN EN ISO 4762 M3 x 12:1 ↔ ISO 4032 M3:1
- Zestawiające:174 [Mate]: YSub1:1 ↔ ISO 4032 M3:1
- [Mate]: DIN EN ISO 4762 M3 x 12:7 ↔ ISO 4032 M3:7
- Zestawiające:176 [Mate]: Cartesian1_X_RodCover:4 ↔ DIN EN ISO 4762 M3 x 12:7
- Zestawiające:177 [Mate]: Cartesian1_X_RodCover:4 ↔ DIN EN ISO 4762 M3 x 12:7
- Zestawiające:178 [Mate]: DIN EN ISO 4762 M3 x 12:7 ↔ ISO 4032 M3:7
- Zestawiające:179 [Mate]: YSub1:1 ↔ ISO 4032 M3:7
- Kątowe:21 [Angle] (0 deg): YSub1:1 ↔ ISO 4032 M3:7
- [Mate]: ISO 4032 M3:13 ↔ DIN EN ISO 4762 M3 x 12:13
- Zestawiające:181 [Mate]: Cartesian1_X_RodCover:1 ↔ DIN EN ISO 4762 M3 x 12:13
- Zestawiające:182 [Mate]: Cartesian1_X_RodCover:1 ↔ DIN EN ISO 4762 M3 x 12:13
- Zestawiające:183 [Mate]: ISO 4032 M3:13 ↔ DIN EN ISO 4762 M3 x 12:13
- Zestawiające:184 [Mate]: YSub2:1 ↔ ISO 4032 M3:13
- Kątowe:22 [Angle] (0 deg): YSub2:1 ↔ ISO 4032 M3:13
- [Mate]: DIN EN ISO 4762 M3 x 12:19 ↔ ISO 4032 M3:19
- Zestawiające:186 [Mate]: Cartesian1_X_RodCover:2 ↔ DIN EN ISO 4762 M3 x 12:19
- Zestawiające:187 [Mate]: Cartesian1_X_RodCover:2 ↔ DIN EN ISO 4762 M3 x 12:19
- Zestawiające:188 [Mate]: YSub2:1 ↔ ISO 4032 M3:19
- Kątowe:23 [Angle] (0 deg): YSub2:1 ↔ ISO 4032 M3:19
- Kątowe:24 [Angle] (0 deg): YSub1:1 ↔ ISO 4032 M3:1
## Named parameters: d253_d246 = 0 mm, d263_d246 = 0 mm, d273_d246 = 0 mm
